# Autodesk Inventor assembly: Motor
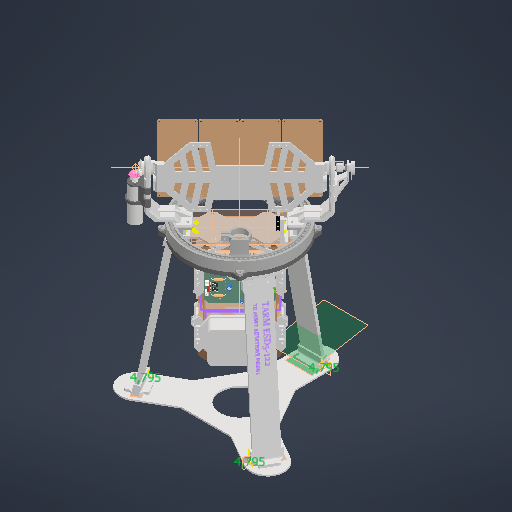
[picture p0: Inventor's stored thumbnail of the model, 512x512]
Saved by Autodesk Inventor 2026.1 (Build 301233020, 233B)
## iProperties
Created: 2025-09-23
Part Number: Motor
Document SubType Name: Assembly
Designer: Malthe Sennels
Author: Malthe Sennels
## Documents named in this file (44)
- C:\Users\Mikke\OneDrive - Aalborg Universitet\ESD 510 - General\Projekt\Inventor\Sentry3\Motor.iam
- C:\Users\Mikke\OneDrive - Aalborg Universitet\ESD 510 - General\Projekt\Inventor\Sentry3\Angle_motor.ipt
- C:\Users\Mikke\OneDrive - Aalborg Universitet\ESD 510 - General\Projekt\Inventor\Sentry3\Bearing.ipt
- C:\Users\Mikke\OneDrive - Aalborg Universitet\ESD 510 - General\Projekt\Inventor\Sentry3\Outer_gear.ipt
- C:\Users\Mikke\OneDrive - Aalborg Universitet\ESD 510 - General\Projekt\Inventor\Sentry3\Inner gear.ipt
- C:\Users\Mikke\OneDrive - Aalborg Universitet\ESD 510 - General\Projekt\Inventor\Sentry3\Motor\Design Accelerator\Spur Gears1.iam
- C:\Users\Mikke\OneDrive - Aalborg Universitet\ESD 510 - General\Projekt\Inventor\Sentry3\Phased_array.ipt
- C:\Users\Mikke\OneDrive - Aalborg Universitet\ESD 510 - General\Projekt\Inventor\Sentry3\Venstre arm.ipt
- C:\Users\Mikke\OneDrive - Aalborg Universitet\ESD 510 - General\Projekt\Inventor\Sentry3\Venstre_rotator.ipt
- C:\Users\Mikke\OneDrive - Aalborg Universitet\ESD 510 - General\Projekt\Inventor\Sentry3\Venstre_bearing_lock.ipt
- C:\Users\Mikke\OneDrive - Aalborg Universitet\ESD 510 - General\Projekt\Inventor\Sentry3\Balls.ipt
- C:\Users\Mikke\OneDrive - Aalborg Universitet\ESD 510 - General\Projekt\Inventor\Sentry3\Motor_elevation.ipt
- C:\Users\Mikke\OneDrive - Aalborg Universitet\ESD 510 - General\Projekt\Inventor\Sentry3\Lazercutlink.ipt
- C:\Users\Mikke\OneDrive - Aalborg Universitet\ESD 510 - General\Projekt\Inventor\Backplane.ipt
- C:\Users\Mikke\OneDrive - Aalborg Universitet\ESD 510 - General\Projekt\Inventor\Sentry3\Motor\Design Accelerator\Bevel Gears1.iam
- C:\Users\Mikke\OneDrive - Aalborg Universitet\ESD 510 - General\Projekt\Inventor\Sentry3\Elevation_mount.ipt
- C:\Users\Mikke\OneDrive - Aalborg Universitet\ESD 510 - General\Projekt\Inventor\Sentry3\Lazercut_base.ipt
- C:\Users\Mikke\OneDrive - Aalborg Universitet\ESD 510 - General\Projekt\Inventor\Sentry3\LEG.ipt
- C:\Users\Mikke\OneDrive - Aalborg Universitet\ESD 510 - General\Projekt\Inventor\Sentry3\Lock buttom.ipt
- C:\Users\Mikke\OneDrive - Aalborg Universitet\ESD 510 - General\Projekt\Inventor\Sentry3\Lysekrone_adapter.ipt
- C:\Users\Mikke\OneDrive - Aalborg Universitet\ESD 510 - General\Projekt\Inventor\Sentry3\Center_lysekrone.ipt
- C:\Users\Mikke\OneDrive - Aalborg Universitet\ESD 510 - General\Projekt\Inventor\Sentry3\USRPB210.ipt
- C:\Users\Mikke\OneDrive - Aalborg Universitet\ESD 510 - General\Projekt\Inventor\Sentry3\RPI.ipt
- C:\Users\Mikke\OneDrive - Aalborg Universitet\ESD 510 - General\Projekt\Inventor\Butler_matrix\Butler_assembly.iam
- C:\Users\Mikke\OneDrive - Aalborg Universitet\ESD 510 - General\Projekt\Inventor\Sentry3\Motor_driver.ipt
- C:\Users\Mikke\OneDrive - Aalborg Universitet\ESD 510 - General\Projekt\Inventor\Sentry3\Krone_interface.ipt
- C:\Users\Mikke\OneDrive - Aalborg Universitet\ESD 510 - General\Projekt\Inventor\Sentry3\Shelf1.ipt
- C:\Users\Mikke\OneDrive - Aalborg Universitet\ESD 510 - General\Projekt\Inventor\Sentry3\Shelf2.ipt
- C:\Users\Mikke\OneDrive - Aalborg Universitet\ESD 510 - General\Projekt\Inventor\Sentry3\RPI_Motordriver_mount.ipt
- C:\Users\Mikke\OneDrive - Aalborg Universitet\ESD 510 - General\Projekt\Inventor\Sentry3\Spacer_1.ipt
- C:\Users\Mikke\OneDrive - Aalborg Universitet\ESD 510 - General\Projekt\Inventor\Sentry3\Spacer_1_MIR.ipt
- C:\Users\Mikke\OneDrive - Aalborg Universitet\ESD 510 - General\Projekt\Inventor\Sentry3\Spacer_1_MIR1.ipt
- C:\Users\Mikke\OneDrive - Aalborg Universitet\ESD 510 - General\Projekt\Inventor\Sentry3\Spacer_1_MIR_MIR.ipt
- C:\Users\Mikke\OneDrive - Aalborg Universitet\ESD 510 - General\Projekt\Inventor\Sentry3\Motordriver_Adapter.ipt
- C:\Users\Mikke\OneDrive - Aalborg Universitet\ESD 510 - General\Projekt\Inventor\Sentry3\Pi_holder.ipt
- C:\Users\Mikke\OneDrive - Aalborg Universitet\ESD 510 - General\Projekt\Inventor\Sentry3\Mux_switch_holder.ipt
- C:\Users\Mikke\OneDrive - Aalborg Universitet\ESD 510 - General\Projekt\Inventor\Mux_pcb.iam
- C:\Users\Mikke\OneDrive - Aalborg Universitet\ESD 510 - General\Projekt\Inventor\Sentry3\Homing_switch_holder.ipt
- C:\Users\Mikke\OneDrive - Aalborg Universitet\ESD 510 - General\Projekt\Inventor\Sentry3\switch.ipt
- C:\Users\Mikke\OneDrive - Aalborg Universitet\ESD 510 - General\Projekt\Inventor\Sentry3\Bund.ipt
- C:\Users\Mikke\OneDrive - Aalborg Universitet\ESD 510 - General\Projekt\Inventor\Sentry3\Pot_holder.ipt
- C:\Users\Mikke\OneDrive - Aalborg Universitet\ESD 510 - General\Projekt\Inventor\Sentry3\Pot_adapter.ipt
- C:\Users\Mikke\OneDrive - Aalborg Universitet\ESD 510 - General\Projekt\Inventor\Sentry3\PotMeter.ipt
- C:\Users\Mikke\OneDrive - Aalborg Universitet\ESD 510 - General\Projekt\Inventor\Sentry3\Potmeter_elemount.ipt
## Components (57 placed, 43 different names)
1. Angle_motor:1
2. Bearing:1 — Flush:2, Flush:3, Flush:4, Flush:5, Flush:7, Flush:8, Flush:11, Mate:2, Flush:21, Flush:22, Flush:23, Flush:24, Flush:30, Mate:7, Mate:8, Mate:9, Flush:41, Mate:26, Mate:27, Mate:28, Mate:29, Mate:30
3. Outer_gear:1 — Flush:3, Flush:37
4. Inner gear:1 — Flush:4, Flush:5
5. Spur Gears:1 [sub-assembly]
6. Phased_array:1 — Flush:11, Flush:12, Flush:13, Flush:14, Flush:15, Flush:16, Flush:17, Flush:18, Flush:19, Flush:20, Symmetry:1
7. Phased_array:2 — Flush:12, Flush:15, Flush:18
8. Phased_array:3 — Flush:13, Flush:16, Flush:19
9. Phased_array:4 — Flush:14, Flush:17, Flush:20, Symmetry:1, Angle:5
10. Venstre arm:1 — Flush:21, Flush:22, Flush:23, Flush:24, Flush:27, Mate:3, Mate:4, Flush:30, Flush:31, Flush:67
11. Venstre_rotator:1 — Mate:4, Flush:31, Mate:17, Mate:18, Mate:19, Flush:65, Mate:47, Mate:48, Mate:49
12. Venstre_bearing_lock:1 — Flush:28, Mate:3
13. Balls:1 — Flush:29
14. Venstre arm:2 — Mate:7, Mate:8, Mate:9, Mate:10, Mate:11, Mate:12, Mate:13, Mate:15, Mate:23, Angle:3, Angle:4, Mate:25
15. Venstre_bearing_lock:2 — Mate:11, Mate:12, Angle:1
16. Balls:2 — Mate:10, Mate:25
17. Motor_elevation:1 — Mate:22, Angle:3, Angle:4, Flush:36
18. Lazercutlink:1 — Flush:34
19. Lazercutlink:2 — Mate:17, Mate:18, Mate:19, Mate:24
20. Backplane:1 — Flush:34, Mate:24, Angle:5
21. Bevel Gears:1 [sub-assembly] — Mate:22, Mate:23
22. Elevation_mount:1 — Flush:36
23. Lysekrone_adapter:1 — Flush:41, Flush:42, Mate:29, Mate:30
24. Lysekrone_adapter:2 — Mate:26, Mate:27, Mate:28
25. Center_lysekrone:1 — Flush:42, Flush:43, Flush:47, Mate:33, Mate:34, Mate:35, Mate:36, Flush:49, Flush:60, Flush:61
26. USRPB210:1 — Flush:43, Flush:46, Flush:48, Flush:49
27. RPI:1 — Mate:41
28. Butler_assembly:1 [sub-assembly] — Mate:37, Flush:55, Flush:56, Flush:59
29. Motor_driver:1 — Flush:46, Mate:38
30. Krone_interface:1 — Flush:47, Mate:33, Mate:34, Mate:35, Mate:36, Flush:48, Flush:50, Flush:51, Flush:55, Mate:38
31. Shelf1:1 — Flush:50, Flush:52
32. Shelf2:1 — Flush:51, Flush:53, Flush:54, Flush:56
33. RPI_Motordriver_mount:1 — Flush:52
34. Spacer_1:1 — Flush:53, Flush:54, Mate:37, Flush:57
35. Spacer_1_MIR:1
36. Spacer_1_MIR1:1
37. Spacer_1_MIR_MIR:1 — Flush:58
38. Motordriver_Adapter:1 — Flush:57
39. Pi_holder:1 — Flush:58, Mate:41
40. Mux_switch_holder:1 — Flush:59, Mate:39, Mate:40
41. Mux_pcb:1 [sub-assembly] — Mate:39, Mate:40
42. Homing_switch_holder:1 — Flush:60, Flush:61, Mate:42, Mate:43
43. switch:1 — Mate:42, Mate:43
44. Bund:1 — Flush:63, Flush:64, Mate:44
45. Pot_holder:1 — Flush:65
46. PotMeter:1 — Mate:50, Mate:51
47. Potmeter_elemount:1 — Flush:67
48. Pot_adapter:1 — Mate:47, Mate:48, Mate:49, Mate:50, Mate:51
49. Lazercut_base:1 — Flush:37
50. Lazercut_base:2 — Flush:38
51. Lazercut_base:3
52. LEG:1 — Flush:38
53. LEG:2
54. LEG:3 — Flush:39, Mate:45, Mate:46
55. Lock buttom:1 — Mate:44, Mate:45, Mate:46
56. Lock buttom:2
57. Lock buttom:3
## Component patterns: (3 elements, first: Lazercut_base:1), (3 elements, first: LEG:1), (3 elements, first: Lock buttom:1)
## Relationships (102: Flush 53, Mate 43, Angle 5, Symmetry 1)
- Flush:2: Bearing:1
- Flush:3 (3 mm): Bearing:1 ↔ Outer_gear:1
- Flush:4: Bearing:1 ↔ Inner gear:1
- Flush:5: Bearing:1 ↔ Inner gear:1
- Flush:7 (-8 mm): Bearing:1
- Flush:8: Bearing:1
- Flush:11 (-10 mm): Bearing:1 ↔ Phased_array:1
- Flush:12: Phased_array:1 ↔ Phased_array:2
- Flush:13: Phased_array:1 ↔ Phased_array:3
- Flush:14: Phased_array:1 ↔ Phased_array:4
- Flush:15: Phased_array:1 ↔ Phased_array:2
- Flush:16: Phased_array:1 ↔ Phased_array:3
- Flush:17: Phased_array:1 ↔ Phased_array:4
- Flush:18 (-61 mm): Phased_array:1 ↔ Phased_array:2
- Flush:19 (-122 mm): Phased_array:1 ↔ Phased_array:3
- Flush:20 (-183 mm): Phased_array:1 ↔ Phased_array:4
- Symmetry:1: Phased_array:1 ↔ Phased_array:4
- Mate:2: Bearing:1
- Flush:21: Bearing:1 ↔ Venstre arm:1
- Flush:22: Bearing:1 ↔ Venstre arm:1
- Flush:23: Bearing:1 ↔ Venstre arm:1
- Flush:24: Bearing:1 ↔ Venstre arm:1
- Flush:27 (0.15 mm): Venstre arm:1
- Flush:28: Venstre_bearing_lock:1
- Mate:3: Venstre arm:1 ↔ Venstre_bearing_lock:1
- Flush:29: Balls:1
- Mate:4: Venstre arm:1 ↔ Venstre_rotator:1
- Flush:30: Bearing:1 ↔ Venstre arm:1
- [Mate]: Venstre arm:2 ↔ Venstre_bearing_lock:2
- Mate:7: Bearing:1 ↔ Venstre arm:2
- Mate:8: Bearing:1 ↔ Venstre arm:2
- Mate:9: Bearing:1 ↔ Venstre arm:2
- Mate:10: Venstre arm:2 ↔ Balls:2
- Mate:11: Venstre arm:2 ↔ Venstre_bearing_lock:2
- Mate:12: Venstre arm:2 ↔ Venstre_bearing_lock:2
- Flush:31: Venstre arm:1 ↔ Venstre_rotator:1
- Mate:13: Venstre arm:2
- Angle:1 (90 deg): Venstre_bearing_lock:2
- Mate:15: Venstre arm:2
- Angle:2 (90 deg)
- Mate:17: Venstre_rotator:1 ↔ Lazercutlink:2
- Mate:18: Venstre_rotator:1 ↔ Lazercutlink:2
- Mate:19: Venstre_rotator:1 ↔ Lazercutlink:2
- Flush:34: Lazercutlink:1 ↔ Backplane:1
- Mate:22: Motor_elevation:1 ↔ Bevel Gears:1
- Mate:23: Venstre arm:2 ↔ Bevel Gears:1
- Angle:3 (90 deg): Venstre arm:2 ↔ Motor_elevation:1
- Angle:4 (90 deg): Venstre arm:2 ↔ Motor_elevation:1
- Flush:36: Motor_elevation:1 ↔ Elevation_mount:1
- Flush:37: Outer_gear:1 ↔ Lazercut_base:1
- Flush:38: Lazercut_base:2 ↔ LEG:1
- Flush:39 (-60 mm): LEG:3
- Mate:24: Lazercutlink:2 ↔ Backplane:1
- Mate:25: Venstre arm:2 ↔ Balls:2
- Angle:5 (180 deg): Phased_array:4 ↔ Backplane:1
- Flush:41: Bearing:1 ↔ Lysekrone_adapter:1
- Mate:26: Bearing:1 ↔ Lysekrone_adapter:2
- Mate:27: Bearing:1 ↔ Lysekrone_adapter:2
- Mate:28: Bearing:1 ↔ Lysekrone_adapter:2
- Flush:42: Lysekrone_adapter:1 ↔ Center_lysekrone:1
- Flush:43 (50 mm): Center_lysekrone:1 ↔ USRPB210:1
- Mate:29: Bearing:1 ↔ Lysekrone_adapter:1
- Mate:30: Bearing:1 ↔ Lysekrone_adapter:1
- Flush:46 (20 mm): USRPB210:1 ↔ Motor_driver:1
- Flush:47: Center_lysekrone:1 ↔ Krone_interface:1
- Mate:33: Center_lysekrone:1 ↔ Krone_interface:1
- Mate:34: Center_lysekrone:1 ↔ Krone_interface:1
- Mate:35: Center_lysekrone:1 ↔ Krone_interface:1
- Mate:36: Center_lysekrone:1 ↔ Krone_interface:1
- Flush:48: USRPB210:1 ↔ Krone_interface:1
- Flush:49: Center_lysekrone:1 ↔ USRPB210:1
- Flush:50: Krone_interface:1 ↔ Shelf1:1
- Flush:51: Krone_interface:1 ↔ Shelf2:1
- Flush:52: Shelf1:1 ↔ RPI_Motordriver_mount:1
- Flush:53: Shelf2:1 ↔ Spacer_1:1
- Flush:54: Shelf2:1 ↔ Spacer_1:1
- Mate:37: Butler_assembly:1 ↔ Spacer_1:1
- Flush:55: Butler_assembly:1 ↔ Krone_interface:1
- Flush:56: Butler_assembly:1 ↔ Shelf2:1
- Flush:57: Spacer_1:1 ↔ Motordriver_Adapter:1
- Mate:38: Motor_driver:1 ↔ Krone_interface:1
- Flush:58: Spacer_1_MIR_MIR:1 ↔ Pi_holder:1
- Flush:59: Butler_assembly:1 ↔ Mux_switch_holder:1
- Mate:39: Mux_switch_holder:1 ↔ Mux_pcb:1
- Mate:40: Mux_switch_holder:1 ↔ Mux_pcb:1
- Mate:41: RPI:1 ↔ Pi_holder:1
- Flush:60: Center_lysekrone:1 ↔ Homing_switch_holder:1
- Flush:61: Center_lysekrone:1 ↔ Homing_switch_holder:1
- Mate:42: Homing_switch_holder:1 ↔ switch:1
- Mate:43: Homing_switch_holder:1 ↔ switch:1
- Flush:63: Bund:1
- Flush:64: Bund:1
- Mate:44: Bund:1 ↔ Lock buttom:1
- Mate:45: LEG:3 ↔ Lock buttom:1
- Mate:46: LEG:3 ↔ Lock buttom:1
- Flush:65: Venstre_rotator:1 ↔ Pot_holder:1
- Flush:67: Venstre arm:1 ↔ Potmeter_elemount:1
- Mate:47: Venstre_rotator:1 ↔ Pot_adapter:1
- Mate:48: Venstre_rotator:1 ↔ Pot_adapter:1
- Mate:49: Venstre_rotator:1 ↔ Pot_adapter:1
- Mate:50: PotMeter:1 ↔ Pot_adapter:1
- Mate:51: PotMeter:1 ↔ Pot_adapter:1
## Named parameters: d48_d43 = 0 mm
